# Autodesk Inventor assembly: Robot Assembly MK2
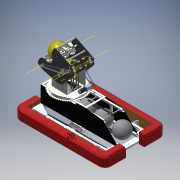
[picture p0: Inventor's stored thumbnail of the model, 180x180]
Saved by Autodesk Inventor 2019.4 (Build 234330000, 330)
## iProperties
Created: 2020-01-18
Part Number: Robot Assembly MK2
Document SubType Name: Assembly
Designer: Mark
Mass: 26362.7 g
Surface Area: 55832.7 cm^2
Volume: 26811.7 cm^3
Density: 0.983254 g/cm^3
Author: Mark
## Documents named in this file (5)
- C:\Users\admin\Desktop\FRC 2020 Engineering\GitHub\7738-2020\Robot Assembly MK2.iam
- C:\Users\admin\Desktop\FRC 2020 Engineering\GitHub\7738-2020\CAD\Drivebase.iam
- C:\Users\admin\Desktop\FRC 2020 Engineering\GitHub\7738-2020\Upper Stage\Upper Stage.iam
- C:\Users\admin\Desktop\FRC 2020 Engineering\GitHub\7738-2020\Robot V2\Turret Columb Assembly\Turret Columb Assembly.iam
- C:\Users\admin\Desktop\FRC 2020 Engineering\GitHub\7738-2020\Robot V2\Bumper\Bumper Half Assembly.iam
## Components (5 placed, 4 different names)
1. Drivebase:1 [sub-assembly] — Mate:1, Flush:1, Flush:2, Mate:4, Mate:5, Mate:6, Mate:7, Flush:4
2. Upper Stage:1 [sub-assembly] — Mate:1, Flush:1, Flush:2, Mate:2, Mate:3
3. Turret Columb Assembly:1 [sub-assembly] — Mate:2, Mate:3
4. Bumper Half Assembly:1 [sub-assembly] — Mate:4, Mate:7, Flush:3, Flush:4
5. Bumper Half Assembly:2 [sub-assembly] — Mate:5, Mate:6, Flush:3
## Relationships (11: Mate 7, Flush 4)
- Mate:1: Drivebase:1 ↔ Upper Stage:1
- Flush:1: Drivebase:1 ↔ Upper Stage:1
- Flush:2: Drivebase:1 ↔ Upper Stage:1
- Mate:2: Upper Stage:1 ↔ Turret Columb Assembly:1
- Mate:3 (0.05 mm): Upper Stage:1 ↔ Turret Columb Assembly:1
- Mate:4: Drivebase:1 ↔ Bumper Half Assembly:1
- Mate:5: Drivebase:1 ↔ Bumper Half Assembly:2
- Mate:6: Drivebase:1 ↔ Bumper Half Assembly:2
- Mate:7: Drivebase:1 ↔ Bumper Half Assembly:1
- Flush:3: Bumper Half Assembly:1 ↔ Bumper Half Assembly:2
- Flush:4 (10 mm): Drivebase:1 ↔ Bumper Half Assembly:1
